# Autodesk Inventor assembly: Assembly2
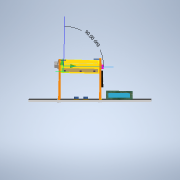
[picture p0: Inventor's stored thumbnail of the model, 180x180]
Saved by Autodesk Inventor 2021 (Build 250183000, 183)
## iProperties
Created: 2021-07-12
Part Number: Assembly2
Document SubType Name: Assembly
Designer: Dell
Author: Dell
## Documents named in this file (18)
- C:\Users\Dell\Desktop\New folder\Assembly2.iam
- C:\Users\Dell\Desktop\Exploration\Maze board\Maze Board 7 (base).ipt
- C:\Users\Dell\Desktop\New folder\1.ipt
- C:\Users\Dell\Desktop\New folder\a1.ipt
- C:\Users\Dell\Desktop\New folder\side.ipt
- C:\Users\Dell\Desktop\New folder\a4.ipt
- C:\Users\Dell\Desktop\Exploration\Maze board\Maze part 4.ipt
- C:\Users\Dell\Documents\Inventor\Content Center Files\R2021\en-US\IFI 502(28)\IFI 502 - 2.2x0.8 x 4(4) AB.ipt
- C:\Users\Dell\Desktop\Exploration\Maze board\pots.ipt
- C:\Users\Dell\Desktop\New folder\18.ipt
- C:\Users\Dell\Desktop\New folder\19.ipt
- C:\Users\Dell\Desktop\New folder\lcd1.ipt
- C:\Users\Dell\Desktop\New folder\lcd2.ipt
- C:\Users\Dell\Desktop\Exploration\Maze board\Maze part 5 (aurdino).ipt
- C:\Users\Dell\Desktop\New folder\bolt.ipt
- C:\Users\Dell\Desktop\New folder\sensor.ipt
- C:\Users\Dell\Desktop\New folder\piezo.ipt
- C:\Users\Dell\Desktop\New folder\rgb led.ipt
## Components (28 placed, 17 different names)
1. Maze Board 7 (base):1 — Flush:1, Mate:1, Mate:2
2. 1:1
3. a1:1 — Angle:1, Angle:2
4. side:1 — Insert:1
5. a4:1 — Angle:1, Angle:2
6. Maze part 4:1
7. Maze part 4:2
8. Indented Hex Flange Head Tapping Screw - Type AB - Metric 2.2x0.8 x 4:1 — Insert:1
9. pots:1
10. pots:2
11. 18:1
12. 18:2
13. 19:1
14. 19:2
15. lcd1:1
16. lcd2:1
17. Maze part 5 (aurdino):1
18. Maze part 5 (aurdino):2
19. bolt:1 — Flush:1
20. bolt:2 — Mate:2
21. bolt:3
22. bolt:4 — Mate:1
23. sensor:1
24. sensor:2
25. sensor:3
26. piezo:1
27. rgb led:1
28. rgb led:2
## Relationships (6: Mate 2, Angle 2, Insert 1, Flush 1)
- Insert:1: side:1 ↔ Indented Hex Flange Head Tapping Screw - Type AB - Metric 2.2x0.8 x 4:1
- Flush:1: Maze Board 7 (base):1 ↔ bolt:1
- Mate:1: Maze Board 7 (base):1 ↔ bolt:4
- Mate:2: Maze Board 7 (base):1 ↔ bolt:2
- Angle:1 (90 deg): a1:1 ↔ a4:1
- Angle:2 (90 deg): a1:1 ↔ a4:1
